# Autodesk Inventor assembly: Boite à musique
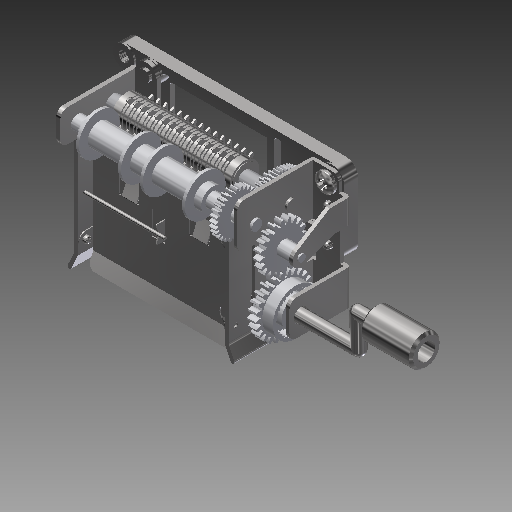
[picture p0: Inventor's stored thumbnail of the model, 512x512]
Saved by Autodesk Inventor 2017 (Build 210142000, 142)
## iProperties
Created: 2016-04-25
Part Number: Boite à musique
Material: Générique
Document SubType Name: Assembly
Designer: Adrien MARY
Stock Number: 1440-02-00
Sending System: Autodesk Translation Framework v4.3.0.3010
Preprocessor: ST-DEVELOPER v16.2
Title: C:/Users/gb9k/Dropbox/Pictures/Music Box/Kikkerland Music Box.step
## Documents named in this file (20)
- W:\Professionnel\Conception FABLAB\1440 Boite a musique\Mecanisme\kikkerland-mechanical-music-box-1.snapshot.3\Inventor\Kikkerland Music Box.iam
- W:\Professionnel\Conception FABLAB\1440 Boite a musique\Mecanisme\kikkerland-mechanical-music-box-1.snapshot.3\Inventor\Bedplate.ipt
- W:\Professionnel\Conception FABLAB\1440 Boite a musique\Mecanisme\kikkerland-mechanical-music-box-1.snapshot.3\Inventor\Right Feeder Tray Support.ipt
- W:\Professionnel\Conception FABLAB\1440 Boite a musique\Mecanisme\kikkerland-mechanical-music-box-1.snapshot.3\Inventor\Comb.ipt
- W:\Professionnel\Conception FABLAB\1440 Boite a musique\Mecanisme\kikkerland-mechanical-music-box-1.snapshot.3\Inventor\Screws.iam
- W:\Professionnel\Conception FABLAB\1440 Boite a musique\Mecanisme\kikkerland-mechanical-music-box-1.snapshot.3\Inventor\Left Feeder Tray Support.ipt
- W:\Professionnel\Conception FABLAB\1440 Boite a musique\Mecanisme\kikkerland-mechanical-music-box-1.snapshot.3\Inventor\Drive Gear Housing.ipt
- W:\Professionnel\Conception FABLAB\1440 Boite a musique\Mecanisme\kikkerland-mechanical-music-box-1.snapshot.3\Inventor\Paper Feed Roller.ipt
- W:\Professionnel\Conception FABLAB\1440 Boite a musique\Mecanisme\kikkerland-mechanical-music-box-1.snapshot.3\Inventor\Feed Gear.ipt
- W:\Professionnel\Conception FABLAB\1440 Boite a musique\Mecanisme\kikkerland-mechanical-music-box-1.snapshot.3\Inventor\Branch Gear 1.ipt
- W:\Professionnel\Conception FABLAB\1440 Boite a musique\Mecanisme\kikkerland-mechanical-music-box-1.snapshot.3\Inventor\Crank Gear.ipt
- W:\Professionnel\Conception FABLAB\1440 Boite a musique\Mecanisme\kikkerland-mechanical-music-box-1.snapshot.3\Inventor\Washers.ipt
- W:\Professionnel\Conception FABLAB\1440 Boite a musique\Mecanisme\kikkerland-mechanical-music-box-1.snapshot.3\Inventor\Drum Plucker.ipt
- W:\Professionnel\Conception FABLAB\1440 Boite a musique\Mecanisme\kikkerland-mechanical-music-box-1.snapshot.3\Inventor\Plucker Gear Sm.ipt
- W:\Professionnel\Conception FABLAB\1440 Boite a musique\Mecanisme\kikkerland-mechanical-music-box-1.snapshot.3\Inventor\Plucker Gear Lg.ipt
- W:\Professionnel\Conception FABLAB\1440 Boite a musique\Mecanisme\kikkerland-mechanical-music-box-1.snapshot.3\Inventor\Branch Gear 2.ipt
- W:\Professionnel\Conception FABLAB\1440 Boite a musique\Mecanisme\kikkerland-mechanical-music-box-1.snapshot.3\Inventor\Lower Feeder Tray.ipt
- W:\Professionnel\Conception FABLAB\1440 Boite a musique\Mecanisme\kikkerland-mechanical-music-box-1.snapshot.3\Inventor\Upper Feeder Tray.ipt
- W:\Professionnel\Conception FABLAB\1440 Boite a musique\Mecanisme\kikkerland-mechanical-music-box-1.snapshot.3\Inventor\Hand Crank.ipt
- W:\Professionnel\Conception FABLAB\1440 Boite a musique\Mecanisme\kikkerland-mechanical-music-box-1.snapshot.3\Inventor\Wire Form.ipt
## Components (19 placed, 19 different names)
1. Bedplate:1
2. Right Feeder Tray Support:1
3. Comb:1
4. Screws:1 [sub-assembly]
5. Left Feeder Tray Support:1
6. Drive Gear Housing:1 — Placage:1, Affleurement:1, Affleurement:2, Affleurement:3, Affleurement:4, Placage:2, Placage:3, Placage:6, Affleurement:5, Affleurement:6, Placage:10
7. Paper Feed Roller:1 — Affleurement:6, Placage:10, Angle:4, Placage:11
8. Feed Gear:1 — Affleurement:4, Angle:4, Placage:11, Rotation:3
9. Branch Gear 1:1 — Affleurement:2, Placage:6, Placage:9, Rotation:1, Angle:2
10. Crank Gear:1 — Affleurement:3, Placage:7, Placage:8, Angle:1, Rotation:1
11. Washers:1
12. Drum Plucker:1 — Placage:4, Placage:5
13. Plucker Gear Sm:1 — Placage:3, Placage:4, Angle:3, Rotation:3
14. Plucker Gear Lg:1 — Placage:2, Placage:5, Angle:3, Rotation:2
15. Branch Gear 2:1 — Affleurement:5, Placage:9, Angle:2, Rotation:2
16. Lower Feeder Tray:1
17. Upper Feeder Tray:1
18. Hand Crank:1 — Placage:1, Affleurement:1, Placage:7, Placage:8, Angle:1, Manivelle
19. Wire Form:1
## Relationships (25: Mate 11, Flush 6, Angle 5, RelateRotation 3)
- Placage:1 [Mate]: Drive Gear Housing:1 ↔ Hand Crank:1
- Affleurement:1 [Flush] (35.54 mm): Drive Gear Housing:1 ↔ Hand Crank:1
- Affleurement:2 [Flush] (4.85 mm): Drive Gear Housing:1 ↔ Branch Gear 1:1
- Affleurement:3 [Flush] (1.5 mm): Drive Gear Housing:1 ↔ Crank Gear:1
- Affleurement:4 [Flush] (4.9 mm): Drive Gear Housing:1 ↔ Feed Gear:1
- Placage:2 [Mate] (0.891 mm): Drive Gear Housing:1 ↔ Plucker Gear Lg:1
- Placage:3 [Mate] (2.841 mm): Drive Gear Housing:1 ↔ Plucker Gear Sm:1
- Placage:4 [Mate]: Drum Plucker:1 ↔ Plucker Gear Sm:1
- Placage:5 [Mate]: Drum Plucker:1 ↔ Plucker Gear Lg:1
- Placage:6 [Mate]: Drive Gear Housing:1 ↔ Branch Gear 1:1
- Placage:7 [Mate]: Crank Gear:1 ↔ Hand Crank:1
- Placage:8 [Mate]: Crank Gear:1 ↔ Hand Crank:1
- Affleurement:5 [Flush] (-2.5 mm): Drive Gear Housing:1 ↔ Branch Gear 2:1
- Placage:9 [Mate]: Branch Gear 1:1 ↔ Branch Gear 2:1
- Affleurement:6 [Flush] (-0.65 mm): Drive Gear Housing:1 ↔ Paper Feed Roller:1
- Placage:10 [Mate]: Drive Gear Housing:1 ↔ Paper Feed Roller:1
- Angle:1 (0 deg): Crank Gear:1 ↔ Hand Crank:1
- Rotation:1 [RelateRotation] (1.25 ul): Branch Gear 1:1 ↔ Crank Gear:1
- Angle:2 (0 deg): Branch Gear 1:1 ↔ Branch Gear 2:1
- Angle:3 (0 deg): Plucker Gear Sm:1 ↔ Plucker Gear Lg:1
- Angle:4 (0 deg): Paper Feed Roller:1 ↔ Feed Gear:1
- Rotation:2 [RelateRotation] (0.1875 ul): Plucker Gear Lg:1 ↔ Branch Gear 2:1
- Placage:11 [Mate]: Paper Feed Roller:1 ↔ Feed Gear:1
- Rotation:3 [RelateRotation] (0.7241 ul): Feed Gear:1 ↔ Plucker Gear Sm:1
- Manivelle [Angle] (17188.7339 deg): Hand Crank:1
